# Autodesk Inventor assembly: машинка
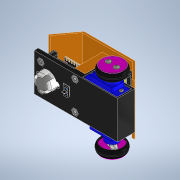
[picture p0: Inventor's stored thumbnail of the model, 180x180]
Saved by Autodesk Inventor 2022 (Build 260153000, 153)
## iProperties
Created: 2025-01-04
Part Number: машинка
Document SubType Name: Assembly
Designer: Admin
Author: Admin
## Documents named in this file (4)
- G:\машина\машинка.iam
- G:\машина\крыша.iam
- G:\машина\крепление.iam
- G:\машина\основа.iam
## Components (3 placed, 3 different names)
1. крыша:1 [sub-assembly]
2. крепление:1 [sub-assembly]
3. основа:1 [sub-assembly]
## Relationships (11: Mate 7, Flush 4)
- [Flush]: основа:1
- [Flush]: основа:1
- [Flush]: основа:1
- [Mate]: крыша:1 ↔ основа:1
- [Mate]: крыша:1 ↔ основа:1
- [Mate]: крыша:1 ↔ основа:1
- [Flush]: крепление:1 ↔ основа:1
- [Mate]: крепление:1 ↔ основа:1
- [Mate]: крепление:1 ↔ основа:1
- [Mate]: крыша:1 ↔ основа:1
- [Mate]: крыша:1 ↔ основа:1
